# Autodesk Inventor assembly: Uptake Assembly
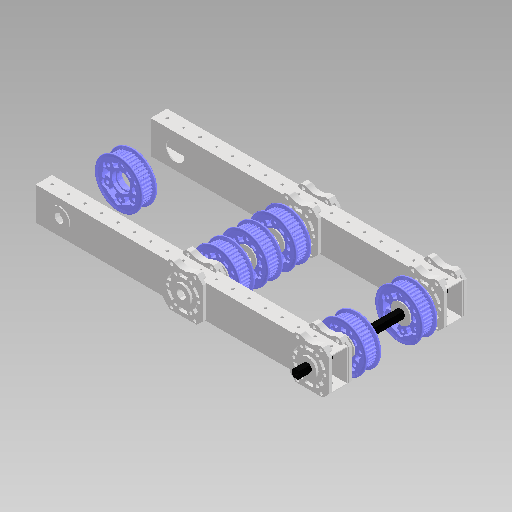
[picture p0: Inventor's stored thumbnail of the model, 512x512]
Saved by Autodesk Inventor 2021 (Build 250183000, 183)
## iProperties
Created: 2021-03-03
Part Number: Uptake Assembly
Document SubType Name: Assembly
Designer: aidan
Author: aidan
## Documents named in this file (7)
- C:\Users\Merkileg\Documents\t3-cad\CAD\2021 Specific Parts\Uptake Assembly.iam
- C:\Users\Merkileg\Documents\t3-cad\CAD\2021 Specific Parts\VerseFrame 18in Uptake.ipt
- C:\Users\Merkileg\Documents\t3-cad\CAD\VersaBlock Assembly.iam
- C:\Users\Merkileg\Documents\t3-cad\CAD\Generic and Stock\am 42 Tooth Pulley Full Shrinkwrap.ipt
- C:\Users\Merkileg\Documents\t3-cad\CAD\10in THUNDERSHAFT.ipt
- C:\Users\Merkileg\Documents\t3-cad\CAD\Generic and Stock\am 42 Tooth Pully with Bearings Shrinkwrap.ipt
- C:\Users\Merkileg\Documents\t3-cad\CAD\Bearing  for THUNDER.ipt
## Components (15 placed, 6 different names)
1. VerseFrame 18in Uptake:1 — Flush:1, Flush:2, Mate:1, Mate:7, Mate:8, Mate:9, Mate:10, Mate:20, Insert:2
2. VerseFrame 18in Uptake:2 — Flush:1, Flush:2, Mate:1, Mate:3, Mate:4, Mate:5, Mate:6, Mate:16, Mate:19, Insert:1, Mate:24, Angle:1, Mate:27, Angle:2
3. VersaBlock Assembly:1 [sub-assembly] — Mate:3, Mate:4, Flush:3, Mate:15, Mate:23, Mate:26
4. VersaBlock Assembly:2 [sub-assembly] — Mate:5, Mate:6, Flush:4, Mate:14, Mate:17, Mate:18, Flush:8, Flush:10
5. VersaBlock Assembly:3 [sub-assembly] — Mate:7, Mate:8, Flush:4
6. VersaBlock Assembly:4 [sub-assembly] — Mate:9, Mate:10, Flush:3
7. am 42 Tooth Pulley Full Shrinkwrap:1 — Mate:16, Flush:5
8. 10in THUNDERSHAFT:1 — Mate:17, Mate:18, Flush:8
9. am 42 Tooth Pully with Bearings Shrinkwrap:1 — Mate:11, Mate:15, Flush:6, Mate:21
10. am 42 Tooth Pully with Bearings Shrinkwrap:2 — Mate:11, Mate:12, Flush:5, Mate:21
11. am 42 Tooth Pully with Bearings Shrinkwrap:3 — Mate:12, Flush:7
12. am 42 Tooth Pully with Bearings Shrinkwrap:4 — Mate:13, Flush:7, Mate:20
13. am 42 Tooth Pully with Bearings Shrinkwrap:5 — Mate:13, Mate:14, Flush:6, Mate:19
14. Bearing  for THUNDER:1 — Insert:1, Flush:9, Mate:22
15. Bearing  for THUNDER:2 — Insert:2, Flush:9
## Relationships (41: Mate 27, Flush 10, Insert 2, Angle 2)
- Flush:1: VerseFrame 18in Uptake:1 ↔ VerseFrame 18in Uptake:2
- Flush:2: VerseFrame 18in Uptake:1 ↔ VerseFrame 18in Uptake:2
- Mate:1 (152.4 mm): VerseFrame 18in Uptake:1 ↔ VerseFrame 18in Uptake:2
- Mate:3: VerseFrame 18in Uptake:2 ↔ VersaBlock Assembly:1
- Mate:4: VerseFrame 18in Uptake:2 ↔ VersaBlock Assembly:1
- Mate:5: VerseFrame 18in Uptake:2 ↔ VersaBlock Assembly:2
- Mate:6: VerseFrame 18in Uptake:2 ↔ VersaBlock Assembly:2
- Mate:7: VerseFrame 18in Uptake:1 ↔ VersaBlock Assembly:3
- Mate:8: VerseFrame 18in Uptake:1 ↔ VersaBlock Assembly:3
- Mate:9: VerseFrame 18in Uptake:1 ↔ VersaBlock Assembly:4
- Mate:10: VerseFrame 18in Uptake:1 ↔ VersaBlock Assembly:4
- Flush:3: VersaBlock Assembly:1 ↔ VersaBlock Assembly:4
- Flush:4: VersaBlock Assembly:2 ↔ VersaBlock Assembly:3
- Mate:11: am 42 Tooth Pully with Bearings Shrinkwrap:1 ↔ am 42 Tooth Pully with Bearings Shrinkwrap:2
- Mate:12: am 42 Tooth Pully with Bearings Shrinkwrap:2 ↔ am 42 Tooth Pully with Bearings Shrinkwrap:3
- Mate:13: am 42 Tooth Pully with Bearings Shrinkwrap:4 ↔ am 42 Tooth Pully with Bearings Shrinkwrap:5
- Mate:14: VersaBlock Assembly:2 ↔ am 42 Tooth Pully with Bearings Shrinkwrap:5
- Mate:15: VersaBlock Assembly:1 ↔ am 42 Tooth Pully with Bearings Shrinkwrap:1
- Mate:16: VerseFrame 18in Uptake:2 ↔ am 42 Tooth Pulley Full Shrinkwrap:1
- Flush:5: am 42 Tooth Pulley Full Shrinkwrap:1 ↔ am 42 Tooth Pully with Bearings Shrinkwrap:2
- Flush:6: am 42 Tooth Pully with Bearings Shrinkwrap:1 ↔ am 42 Tooth Pully with Bearings Shrinkwrap:5
- Flush:7: am 42 Tooth Pully with Bearings Shrinkwrap:3 ↔ am 42 Tooth Pully with Bearings Shrinkwrap:4
- Mate:17: VersaBlock Assembly:2 ↔ 10in THUNDERSHAFT:1
- Mate:18: VersaBlock Assembly:2 ↔ 10in THUNDERSHAFT:1
- Flush:8 (17.4498 mm): VersaBlock Assembly:2 ↔ 10in THUNDERSHAFT:1
- Mate:19 (25.4 mm): VerseFrame 18in Uptake:2 ↔ am 42 Tooth Pully with Bearings Shrinkwrap:5
- Mate:20 (25.4 mm): VerseFrame 18in Uptake:1 ↔ am 42 Tooth Pully with Bearings Shrinkwrap:4
- Mate:21 (28.8544 mm): am 42 Tooth Pully with Bearings Shrinkwrap:1 ↔ am 42 Tooth Pully with Bearings Shrinkwrap:2
- Insert:1: VerseFrame 18in Uptake:2 ↔ Bearing  for THUNDER:1
- Insert:2: VerseFrame 18in Uptake:1 ↔ Bearing  for THUNDER:2
- Flush:9: Bearing  for THUNDER:1 ↔ Bearing  for THUNDER:2
- Mate:22: Bearing  for THUNDER:1
- Mate:23: VersaBlock Assembly:1
- Mate:24: VerseFrame 18in Uptake:2
- Mate:25
- Angle:1 (0 deg): VerseFrame 18in Uptake:2
- Mate:26 (-30.5181 mm): VersaBlock Assembly:1
- Mate:27: VerseFrame 18in Uptake:2
- Mate:28
- Angle:2 (0 deg): VerseFrame 18in Uptake:2
- Flush:10 (-30.5181 mm): VersaBlock Assembly:2
